# Autodesk Inventor assembly: piston_Assembly
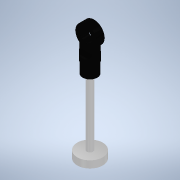
[picture p0: Inventor's stored thumbnail of the model, 180x180]
Saved by Autodesk Inventor 2020.2 (Build 242310000, 310)
## iProperties
Created: 2019-12-06
Part Number: piston_Assembly
Document SubType Name: Assembly
Designer: axelj
Author: axelj
## Documents named in this file (3)
- C:\Users\axelj\OneDrive\Documentos\GitHub\autobot\robot_model\piston_Assembly.iam
- C:\Users\axelj\OneDrive\Documentos\GitHub\autobot\robot_model\RCT-T005_Embolo.ipt
- C:\Users\axelj\OneDrive\Documentos\GitHub\autobot\robot_model\RCT-T005_Conexion_superioript.ipt
## Components (2 placed, 2 different names)
1. RCT-T005_Embolo:1 — Coincidencia:1
2. RCT-T005_Conexion_superioript:1 — Coincidencia:1
## Relationships (1: Mate 1)
- Coincidencia:1 [Mate]: RCT-T005_Embolo:1 ↔ RCT-T005_Conexion_superioript:1
